# Autodesk Inventor assembly: all_body
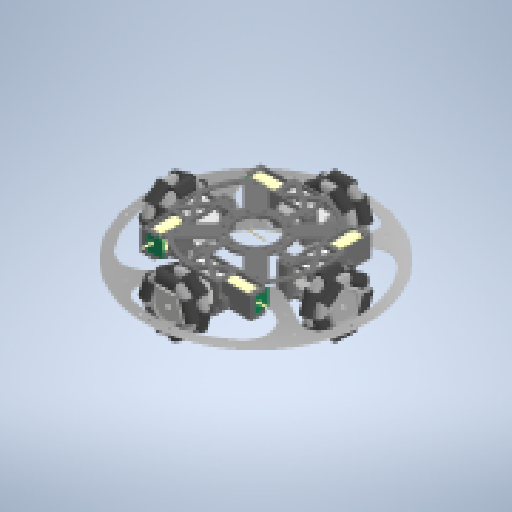
[picture p0: Inventor's stored thumbnail of the model, 512x512]
Saved by Autodesk Inventor 2024.1 (Build 281209000, 209)
## iProperties
Created: 2024-08-02
Part Number: all_body
Document SubType Name: Assembly
Designer: hibik
Author: hibik
## Documents named in this file (8)
- C:\Users\hibik\Desktop\ロボメカ\Rescue\2年\子機_本選\body_locom.iam
- C:\Users\hibik\Desktop\ロボメカ\Rescue\2年\子機_本選\body_upper.ipt
- C:\Users\hibik\Desktop\ロボメカ\Rescue\2年\子機_本選\body_under.ipt
- C:\Users\hibik\Desktop\ロボメカ\Rescue\2年\子機_本選\Motor.ipt
- C:\Users\hibik\Desktop\ロボメカ\Rescue\2年\子機_本選\omni.iam
- C:\Users\hibik\Desktop\ロボメカ\Rescue\2年\子機_本選\Motor_400.ipt
- C:\Users\hibik\Desktop\ロボメカ\Rescue\2年\子機_本選\encoder.ipt
- C:\Users\hibik\Desktop\ロボメカ\Rescue\2年\子機_本選\body_plate.ipt
## Components (25 placed, 7 different names)
1. body_upper:1 — 挿入:1, 挿入:2, 挿入:3, 挿入:4, フラッシュ:1, フラッシュ:2, フラッシュ:3, フラッシュ:4, メイト:1, メイト:2, メイト:3, メイト:4, メイト:5, メイト:6, メイト:7, メイト:8, メイト:9, メイト:10, メイト:11, メイト:12, 挿入:9, 挿入:10, 挿入:11, 挿入:12, 角度:1, 角度:2, 角度:3, 角度:4, 挿入:13, 挿入:14, 挿入:15, 挿入:16, 角度:5, 角度:6, 角度:7, 角度:8, 挿入:17, 挿入:18
2. body_under:1 — 挿入:1, フラッシュ:2
3. body_under:2 — 挿入:4, フラッシュ:1
4. body_under:3 — 挿入:3, フラッシュ:4
5. body_under:4 — 挿入:2, フラッシュ:3
6. Motor:1 — メイト:1, メイト:6, メイト:10, 挿入:5
7. Motor:2 — メイト:2, メイト:7, メイト:11, 挿入:8
8. Motor:3 — メイト:3, メイト:8, メイト:9, 挿入:7
9. Motor:4 — メイト:4, メイト:5, メイト:12, 挿入:6
10. omni:1 [sub-assembly] — 挿入:8
11. omni:2 [sub-assembly] — 挿入:7
12. omni:3 [sub-assembly] — 挿入:6
13. omni:4 [sub-assembly] — 挿入:5
14. Motor_400:1 — 挿入:12, 角度:1
15. Motor_400:2 — 挿入:11, 角度:4
16. Motor_400:3 — 挿入:9, 角度:2
17. Motor_400:4 — 挿入:10, 角度:3
18. encoder:1 — 挿入:13, 角度:6
19. encoder:2 — 挿入:14, 角度:7
20. encoder:3 — 挿入:15, 角度:8
21. encoder:4 — 挿入:16, 角度:5
22. body_plate:2 — 挿入:19, 挿入:20, 挿入:21, メイト:14, メイト:15
23. body_plate:3 — 挿入:20, メイト:13
24. body_plate:4 — 挿入:21, メイト:14
25. body_plate:5 — 挿入:17, 挿入:18, 挿入:19, メイト:13, メイト:15
## Relationships (48: Insert 21, Mate 15, Angle 8, Flush 4)
- 挿入:1 [Insert]: body_upper:1 ↔ body_under:1
- 挿入:2 [Insert]: body_upper:1 ↔ body_under:4
- 挿入:3 [Insert]: body_upper:1 ↔ body_under:3
- 挿入:4 [Insert]: body_upper:1 ↔ body_under:2
- フラッシュ:1 [Flush]: body_upper:1 ↔ body_under:2
- フラッシュ:2 [Flush]: body_upper:1 ↔ body_under:1
- フラッシュ:3 [Flush]: body_upper:1 ↔ body_under:4
- フラッシュ:4 [Flush]: body_upper:1 ↔ body_under:3
- メイト:1 [Mate]: body_upper:1 ↔ Motor:1
- メイト:2 [Mate]: body_upper:1 ↔ Motor:2
- メイト:3 [Mate]: body_upper:1 ↔ Motor:3
- メイト:4 [Mate]: body_upper:1 ↔ Motor:4
- メイト:5 [Mate]: body_upper:1 ↔ Motor:4
- メイト:6 [Mate]: body_upper:1 ↔ Motor:1
- メイト:7 [Mate]: body_upper:1 ↔ Motor:2
- メイト:8 [Mate]: body_upper:1 ↔ Motor:3
- メイト:9 [Mate]: body_upper:1 ↔ Motor:3
- メイト:10 [Mate]: body_upper:1 ↔ Motor:1
- メイト:11 [Mate]: body_upper:1 ↔ Motor:2
- メイト:12 [Mate]: body_upper:1 ↔ Motor:4
- 挿入:5 [Insert]: Motor:1 ↔ omni:4
- 挿入:6 [Insert]: Motor:4 ↔ omni:3
- 挿入:7 [Insert]: Motor:3 ↔ omni:2
- 挿入:8 [Insert]: Motor:2 ↔ omni:1
- 挿入:9 [Insert]: body_upper:1 ↔ Motor_400:3
- 挿入:10 [Insert]: body_upper:1 ↔ Motor_400:4
- 挿入:11 [Insert]: body_upper:1 ↔ Motor_400:2
- 挿入:12 [Insert]: body_upper:1 ↔ Motor_400:1
- 角度:1 [Angle] (0 deg): body_upper:1 ↔ Motor_400:1
- 角度:2 [Angle] (0 deg): body_upper:1 ↔ Motor_400:3
- 角度:3 [Angle] (0 deg): body_upper:1 ↔ Motor_400:4
- 角度:4 [Angle] (0 deg): body_upper:1 ↔ Motor_400:2
- 挿入:13 [Insert]: body_upper:1 ↔ encoder:1
- 挿入:14 [Insert]: body_upper:1 ↔ encoder:2
- 挿入:15 [Insert]: body_upper:1 ↔ encoder:3
- 挿入:16 [Insert]: body_upper:1 ↔ encoder:4
- 角度:5 [Angle] (0 deg): body_upper:1 ↔ encoder:4
- 角度:6 [Angle] (0 deg): body_upper:1 ↔ encoder:1
- 角度:7 [Angle] (0 deg): body_upper:1 ↔ encoder:2
- 角度:8 [Angle] (0 deg): body_upper:1 ↔ encoder:3
- 挿入:17 [Insert]: body_upper:1 ↔ body_plate:5
- 挿入:18 [Insert]: body_upper:1 ↔ body_plate:5
- 挿入:19 [Insert]: body_plate:2 ↔ body_plate:5
- 挿入:20 [Insert]: body_plate:2 ↔ body_plate:3
- 挿入:21 [Insert]: body_plate:2 ↔ body_plate:4
- メイト:13 [Mate]: body_plate:3 ↔ body_plate:5
- メイト:14 [Mate]: body_plate:2 ↔ body_plate:4
- メイト:15 [Mate]: body_plate:2 ↔ body_plate:5
